# Autodesk Inventor assembly: 5A.00.02.01-IB-VTP-Final-Master-Assy
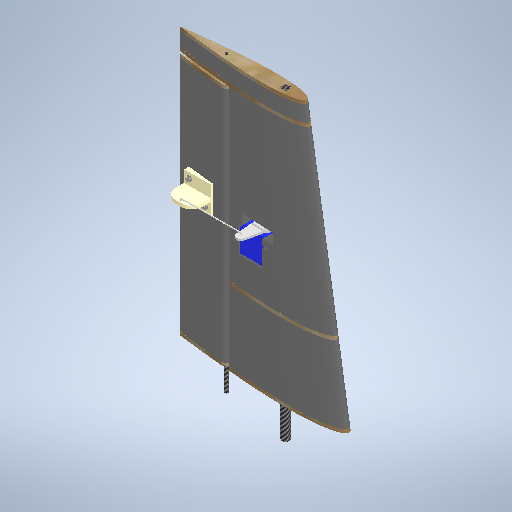
[picture p0: Inventor's stored thumbnail of the model, 512x512]
Saved by Autodesk Inventor 2025.2 (Build 292293000, 293)
## iProperties
Created: 2025-01-14
Part Number: 5A.00.02.01-IB-VTP-Final-Master-Assy
Document SubType Name: Assembly
Designer: inigo
Author: inigo
## Documents named in this file (27)
- C:\Users\inigo\OneDrive - University of Bristol\General - grp-Company A - AVDASI2 2024-25\Full Assembly\VTP\5A.00.02.01-IB-VTP-Final-Master-Assy.iam
- C:\Users\inigo\OneDrive - University of Bristol\General - grp-Company A - AVDASI2 2024-25\Full Assembly\VTP\5P.00.06.01-IB-VTP-Main-Spar.ipt
- C:\Users\inigo\OneDrive - University of Bristol\General - grp-Company A - AVDASI2 2024-25\Full Assembly\VTP\5P.00.08.01-IB-Rear-Spar.ipt
- C:\Users\inigo\OneDrive - University of Bristol\General - grp-Company A - AVDASI2 2024-25\Full Assembly\VTP\EMAX-09-MD Servo.ipt
- C:\Users\inigo\OneDrive - University of Bristol\General - grp-Company A - AVDASI2 2024-25\Full Assembly\VTP\5P.00.02.01-IB-VTP-Body-Final-Right-Second-Rib.ipt
- C:\Users\inigo\OneDrive - University of Bristol\General - grp-Company A - AVDASI2 2024-25\Full Assembly\VTP\5P.00.24.01-IB-VTP-Body-Final-Right-Top.ipt
- C:\Users\inigo\OneDrive - University of Bristol\General - grp-Company A - AVDASI2 2024-25\Full Assembly\VTP\5P.00.10.01-IB-VTP-Body-Final-Right-Main.ipt
- C:\Users\inigo\OneDrive - University of Bristol\General - grp-Company A - AVDASI2 2024-25\Full Assembly\VTP\5P.00.09.01-IB-VTP-Body-Final-Right-Bottom.ipt
- C:\Users\inigo\OneDrive - University of Bristol\General - grp-Company A - AVDASI2 2024-25\Full Assembly\VTP\5P.00.11.01-IB-VTP-Body-Final-Top-Rib.ipt
- C:\Users\inigo\OneDrive - University of Bristol\General - grp-Company A - AVDASI2 2024-25\Full Assembly\VTP\5P.00.12.01-IB-VTP-Body-Final-Middle-Rib.ipt
- C:\Users\inigo\OneDrive - University of Bristol\General - grp-Company A - AVDASI2 2024-25\Full Assembly\VTP\5P.00.13.01-IB-VTP-Body-Final-Bottom-Rib.ipt
- C:\Users\inigo\OneDrive - University of Bristol\General - grp-Company A - AVDASI2 2024-25\Full Assembly\VTP\5P.00.14.01-IB-VTP-Body-Final-Left-Top.ipt
- C:\Users\inigo\OneDrive - University of Bristol\General - grp-Company A - AVDASI2 2024-25\Full Assembly\VTP\5P.00.15.01-IB-VTP-Body-Final-Left-Bottom.ipt
- C:\Users\inigo\OneDrive - University of Bristol\General - grp-Company A - AVDASI2 2024-25\Full Assembly\VTP\5P.00.16.01-IB-VTP-Body-Final-Left-Main.ipt
- C:\Users\inigo\OneDrive - University of Bristol\General - grp-Company A - AVDASI2 2024-25\Full Assembly\VTP\5P.00.04.01-IB-VTP-Rudder-Right.ipt
- C:\Users\inigo\OneDrive - University of Bristol\General - grp-Company A - AVDASI2 2024-25\Full Assembly\VTP\5P.00.07.01-IB-VTP-Rudder-Bottom-Rib.ipt
- C:\Users\inigo\OneDrive - University of Bristol\General - grp-Company A - AVDASI2 2024-25\Full Assembly\VTP\5P.00.05.01-IB-VTP-Rudder-Left.ipt
- C:\Users\inigo\OneDrive - University of Bristol\General - grp-Company A - AVDASI2 2024-25\Full Assembly\VTP\5P.00.18.01-IB-VTP-Rudder-Top-Rib.ipt
- C:\Users\inigo\OneDrive - University of Bristol\General - grp-Company A - AVDASI2 2024-25\Full Assembly\VTP\5P.00.17.01-IB-VTP-Control-Horn.ipt
- C:\Users\inigo\OneDrive - University of Bristol\General - grp-Company A - AVDASI2 2024-25\Full Assembly\VTP\5P.00.19.01-IB-VTP-Servo-Horn.ipt
- C:\Users\inigo\OneDrive - University of Bristol\General - grp-Company A - AVDASI2 2024-25\Full Assembly\VTP\5P.00.20.01-IB-VTP-Control-Rod.ipt
- C:\Users\inigo\OneDrive - University of Bristol\General - grp-Company A - AVDASI2 2024-25\Full Assembly\VTP\5P.00.21.01-IB-VTP-Rudder-Backplate.ipt
- C:\Users\inigo\OneDrive - University of Bristol\General - grp-Company A - AVDASI2 2024-25\Full Assembly\VTP\5P.00.23.01-IB-VTP-Servo-Rear-Retaining-Rod.ipt
- C:\Users\inigo\OneDrive - University of Bristol\General - grp-Company A - AVDASI2 2024-25\Full Assembly\VTP\5P.00.22.01-IB-VTP-Servo-Front-Retaining-Rod.ipt
- C:\Users\inigo\Documents\Inventor\Content Center Files\R2024\en-US\ISO 4762(2)\ISO 4762 - M2 x 16ISO.ipt
- C:\Users\inigo\Documents\Inventor\Content Center Files\R2024\en-US\ISO 7089\ISO 7089 - 2 - 140 HV(1).ipt
- C:\Users\inigo\Documents\Inventor\Content Center Files\R2024\en-US\ISO 4032(2)\ISO 4032 - M2 - ISO.ipt
## Components (31 placed, 26 different names)
1. 5P.00.06.01-IB-VTP-Main-Spar:1 — Mate:1, Flush:1, Mate:3, Mate:6, Mate:9, Mate:12, Mate:14, Mate:16, Mate:18, Mate:20, Mate:29, Mate:51
2. 5P.00.08.01-IB-Rear-Spar:1 — Mate:2, Flush:2, Mate:4, Mate:7, Mate:10, Mate:31, Mate:33, Mate:35, Mate:37
3. EMAX-09-MD Servo:1 — Mate:22, Mate:23, Mate:24, Mate:25, Mate:27, Mate:48, Mate:49
4. 5P.00.02.01-IB-VTP-Body-Final-Second-Rib:1 — Mate:9, Mate:10, Mate:32, Mate:54, Mate:55, Mate:56
5. 5P.00.24.01-IB-VTP-Body-Final-Right-Top:1 — Mate:6, Mate:7, Mate:57, Mate:75
6. 5P.00.09.01-IB-VTP-Body-Final-Right-Bottom:1 — Mate:20, Mate:21, Mate:52
7. 5P.00.11.01-IB-VTP-Body-Final-Top-Rib:1 — Mate:1, Mate:2, Flush:1, Flush:2, Mate:74, Mate:75
8. 5P.00.12.01-IB-VTP-Body-Final-Middle-Rib:1 — Mate:14, Flush:3, Mate:15, Mate:17, Mate:21
9. 5P.00.13.01-IB-VTP-Body-Final-Bottom-Rib:1 — Mate:18, Mate:19, Flush:5
10. 5P.00.14.01-IB-VTP-Body-Final-Left-Top:1 — Mate:3, Mate:4, Mate:54, Angle:1, Mate:74
11. 5P.00.15.01-IB-VTP-Body-Final-Left-Bottom:1 — Mate:16, Flush:4, Mate:17, Mate:19, Flush:5, Mate:52
12. 5P.00.10.01-IB-VTP-Body-Final-Right-Main:1 — Mate:29, Flush:6, Mate:55
13. 5P.00.16.01-IB-VTP-Body-Final-Left-Main:1 — Mate:12, Flush:3, Mate:15, Flush:4, Mate:22, Mate:23, Mate:24, Mate:26, Mate:28, Flush:6, Mate:56, Angle:1
14. 5P.00.04.01-IB-VTP-Rudder-Right:1 — Mate:35, Mate:36, Mate:38, Mate:41, Mate:42, Mate:43, Mate:53
15. 5P.00.07.01-IB-VTP-Rudder-Bottom-Rib:1 — Mate:37, Mate:38, Mate:39
16. 5P.00.05.01-IB-VTP-Rudder-Left:1 — Mate:33, Mate:34, Mate:39, Mate:40, Mate:44, Mate:45, Mate:46, Mate:53
17. 5P.00.18.01-IB-VTP-Rudder-Top-Rib:1 — Mate:31, Mate:32, Mate:34, Mate:36, Mate:40
18. 5P.00.17.01-IB-VTP-Control-Horn:1 — Mate:41, Mate:42, Mate:43, Mate:47, Flush:7, Mate:62, Mate:63, Mate:64, Mate:65
19. 5P.00.20.01-IB-VTP-Control-Rod:1 — Mate:47, Mate:50, Flush:7
20. 5P.00.21.01-IB-VTP-Rudder-Backplate:1 — Mate:44, Mate:45, Mate:46, Mate:67, Mate:69
21. 5P.00.23.01-IB-VTP-Servo-Rear-Retaining-Rod:1 — Mate:25, Mate:26
22. 5P.00.22.01-IB-VTP-Servo-Front-Retaining-Rod:1 — Mate:27, Mate:28
23. 5P.00.19.01-IB-VTP-Servo-Horn:1 — Mate:48, Mate:49, Mate:50
24. ISO 4762 M2 x 16:1 — Mate:58, Mate:59, Mate:64, Mate:66, Mate:70
25. ISO 7089 2:1 — Mate:58, Mate:59, Mate:65
26. ISO 4762 M2 x 16:2 — Mate:62, Mate:68, Mate:72
27. ISO 7089 2:2 — Mate:63
28. ISO 7089 2:3 — Mate:66, Mate:67, Mate:71
29. ISO 7089 2:4 — Mate:68, Mate:69, Mate:73
30. ISO 4032 M2:1 — Mate:70, Mate:71
31. ISO 4032 M2:2 — Mate:72, Mate:73
## Relationships (78: Mate 70, Flush 7, Angle 1)
- Mate:1: 5P.00.06.01-IB-VTP-Main-Spar:1 ↔ 5P.00.11.01-IB-VTP-Body-Final-Top-Rib:1
- Mate:2: 5P.00.08.01-IB-Rear-Spar:1 ↔ 5P.00.11.01-IB-VTP-Body-Final-Top-Rib:1
- Flush:1: 5P.00.06.01-IB-VTP-Main-Spar:1 ↔ 5P.00.11.01-IB-VTP-Body-Final-Top-Rib:1
- Flush:2: 5P.00.08.01-IB-Rear-Spar:1 ↔ 5P.00.11.01-IB-VTP-Body-Final-Top-Rib:1
- Mate:3: 5P.00.06.01-IB-VTP-Main-Spar:1 ↔ 5P.00.14.01-IB-VTP-Body-Final-Left-Top:1
- Mate:4: 5P.00.08.01-IB-Rear-Spar:1 ↔ 5P.00.14.01-IB-VTP-Body-Final-Left-Top:1
- Mate:6: 5P.00.06.01-IB-VTP-Main-Spar:1 ↔ 5P.00.24.01-IB-VTP-Body-Final-Right-Top:1
- Mate:7: 5P.00.08.01-IB-Rear-Spar:1 ↔ 5P.00.24.01-IB-VTP-Body-Final-Right-Top:1
- Mate:9: 5P.00.06.01-IB-VTP-Main-Spar:1 ↔ 5P.00.02.01-IB-VTP-Body-Final-Second-Rib:1
- Mate:10: 5P.00.08.01-IB-Rear-Spar:1 ↔ 5P.00.02.01-IB-VTP-Body-Final-Second-Rib:1
- Mate:12: 5P.00.06.01-IB-VTP-Main-Spar:1 ↔ 5P.00.16.01-IB-VTP-Body-Final-Left-Main:1
- Mate:14: 5P.00.06.01-IB-VTP-Main-Spar:1 ↔ 5P.00.12.01-IB-VTP-Body-Final-Middle-Rib:1
- Flush:3: 5P.00.12.01-IB-VTP-Body-Final-Middle-Rib:1 ↔ 5P.00.16.01-IB-VTP-Body-Final-Left-Main:1
- Mate:15: 5P.00.12.01-IB-VTP-Body-Final-Middle-Rib:1 ↔ 5P.00.16.01-IB-VTP-Body-Final-Left-Main:1
- Mate:16: 5P.00.06.01-IB-VTP-Main-Spar:1 ↔ 5P.00.15.01-IB-VTP-Body-Final-Left-Bottom:1
- Flush:4: 5P.00.15.01-IB-VTP-Body-Final-Left-Bottom:1 ↔ 5P.00.16.01-IB-VTP-Body-Final-Left-Main:1
- Mate:17: 5P.00.12.01-IB-VTP-Body-Final-Middle-Rib:1 ↔ 5P.00.15.01-IB-VTP-Body-Final-Left-Bottom:1
- Mate:18: 5P.00.06.01-IB-VTP-Main-Spar:1 ↔ 5P.00.13.01-IB-VTP-Body-Final-Bottom-Rib:1
- Mate:19: 5P.00.13.01-IB-VTP-Body-Final-Bottom-Rib:1 ↔ 5P.00.15.01-IB-VTP-Body-Final-Left-Bottom:1
- Flush:5: 5P.00.13.01-IB-VTP-Body-Final-Bottom-Rib:1 ↔ 5P.00.15.01-IB-VTP-Body-Final-Left-Bottom:1
- Mate:20: 5P.00.06.01-IB-VTP-Main-Spar:1 ↔ 5P.00.09.01-IB-VTP-Body-Final-Right-Bottom:1
- Mate:21: 5P.00.09.01-IB-VTP-Body-Final-Right-Bottom:1 ↔ 5P.00.12.01-IB-VTP-Body-Final-Middle-Rib:1
- Mate:22: EMAX-09-MD Servo:1 ↔ 5P.00.16.01-IB-VTP-Body-Final-Left-Main:1
- Mate:23: EMAX-09-MD Servo:1 ↔ 5P.00.16.01-IB-VTP-Body-Final-Left-Main:1
- Mate:24: EMAX-09-MD Servo:1 ↔ 5P.00.16.01-IB-VTP-Body-Final-Left-Main:1
- Mate:25: EMAX-09-MD Servo:1 ↔ 5P.00.23.01-IB-VTP-Servo-Rear-Retaining-Rod:1
- Mate:26: 5P.00.16.01-IB-VTP-Body-Final-Left-Main:1 ↔ 5P.00.23.01-IB-VTP-Servo-Rear-Retaining-Rod:1
- Mate:27: EMAX-09-MD Servo:1 ↔ 5P.00.22.01-IB-VTP-Servo-Front-Retaining-Rod:1
- Mate:28: 5P.00.16.01-IB-VTP-Body-Final-Left-Main:1 ↔ 5P.00.22.01-IB-VTP-Servo-Front-Retaining-Rod:1
- Mate:29: 5P.00.06.01-IB-VTP-Main-Spar:1 ↔ 5P.00.10.01-IB-VTP-Body-Final-Right-Main:1
- Flush:6: 5P.00.10.01-IB-VTP-Body-Final-Right-Main:1 ↔ 5P.00.16.01-IB-VTP-Body-Final-Left-Main:1
- Mate:31: 5P.00.08.01-IB-Rear-Spar:1 ↔ 5P.00.18.01-IB-VTP-Rudder-Top-Rib:1
- Mate:32 (2 mm): 5P.00.02.01-IB-VTP-Body-Final-Second-Rib:1 ↔ 5P.00.18.01-IB-VTP-Rudder-Top-Rib:1
- Mate:33: 5P.00.08.01-IB-Rear-Spar:1 ↔ 5P.00.05.01-IB-VTP-Rudder-Left:1
- Mate:34: 5P.00.05.01-IB-VTP-Rudder-Left:1 ↔ 5P.00.18.01-IB-VTP-Rudder-Top-Rib:1
- Mate:35: 5P.00.08.01-IB-Rear-Spar:1 ↔ 5P.00.04.01-IB-VTP-Rudder-Right:1
- Mate:36: 5P.00.04.01-IB-VTP-Rudder-Right:1 ↔ 5P.00.18.01-IB-VTP-Rudder-Top-Rib:1
- Mate:37: 5P.00.08.01-IB-Rear-Spar:1 ↔ 5P.00.07.01-IB-VTP-Rudder-Bottom-Rib:1
- Mate:38: 5P.00.04.01-IB-VTP-Rudder-Right:1 ↔ 5P.00.07.01-IB-VTP-Rudder-Bottom-Rib:1
- Mate:39: 5P.00.07.01-IB-VTP-Rudder-Bottom-Rib:1 ↔ 5P.00.05.01-IB-VTP-Rudder-Left:1
- Mate:40: 5P.00.05.01-IB-VTP-Rudder-Left:1 ↔ 5P.00.18.01-IB-VTP-Rudder-Top-Rib:1
- Mate:41: 5P.00.04.01-IB-VTP-Rudder-Right:1 ↔ 5P.00.17.01-IB-VTP-Control-Horn:1
- Mate:42: 5P.00.04.01-IB-VTP-Rudder-Right:1 ↔ 5P.00.17.01-IB-VTP-Control-Horn:1
- Mate:43 (-6 mm): 5P.00.04.01-IB-VTP-Rudder-Right:1 ↔ 5P.00.17.01-IB-VTP-Control-Horn:1
- Mate:44: 5P.00.05.01-IB-VTP-Rudder-Left:1 ↔ 5P.00.21.01-IB-VTP-Rudder-Backplate:1
- Mate:45 (-6 mm): 5P.00.05.01-IB-VTP-Rudder-Left:1 ↔ 5P.00.21.01-IB-VTP-Rudder-Backplate:1
- Mate:46: 5P.00.05.01-IB-VTP-Rudder-Left:1 ↔ 5P.00.21.01-IB-VTP-Rudder-Backplate:1
- Mate:47: 5P.00.17.01-IB-VTP-Control-Horn:1 ↔ 5P.00.20.01-IB-VTP-Control-Rod:1
- Mate:48: EMAX-09-MD Servo:1 ↔ 5P.00.19.01-IB-VTP-Servo-Horn:1
- Mate:49: EMAX-09-MD Servo:1 ↔ 5P.00.19.01-IB-VTP-Servo-Horn:1
- Mate:50: 5P.00.20.01-IB-VTP-Control-Rod:1 ↔ 5P.00.19.01-IB-VTP-Servo-Horn:1
- Flush:7 (-1 mm): 5P.00.17.01-IB-VTP-Control-Horn:1 ↔ 5P.00.20.01-IB-VTP-Control-Rod:1
- Mate:51: 5P.00.06.01-IB-VTP-Main-Spar:1
- Mate:52: 5P.00.09.01-IB-VTP-Body-Final-Right-Bottom:1 ↔ 5P.00.15.01-IB-VTP-Body-Final-Left-Bottom:1
- Mate:53: 5P.00.04.01-IB-VTP-Rudder-Right:1 ↔ 5P.00.05.01-IB-VTP-Rudder-Left:1
- Mate:54: 5P.00.02.01-IB-VTP-Body-Final-Second-Rib:1 ↔ 5P.00.14.01-IB-VTP-Body-Final-Left-Top:1
- Mate:55: 5P.00.02.01-IB-VTP-Body-Final-Second-Rib:1 ↔ 5P.00.10.01-IB-VTP-Body-Final-Right-Main:1
- Mate:56: 5P.00.02.01-IB-VTP-Body-Final-Second-Rib:1 ↔ 5P.00.16.01-IB-VTP-Body-Final-Left-Main:1
- Angle:1 (90 deg): 5P.00.14.01-IB-VTP-Body-Final-Left-Top:1 ↔ 5P.00.16.01-IB-VTP-Body-Final-Left-Main:1
- Mate:57: 5P.00.24.01-IB-VTP-Body-Final-Right-Top:1
- Mate:58: ISO 4762 M2 x 16:1 ↔ ISO 7089 2:1
- Mate:59: ISO 4762 M2 x 16:1 ↔ ISO 7089 2:1
- [Mate]: ISO 4762 M2 x 16:2 ↔ ISO 7089 2:2
- [Mate]: ISO 4762 M2 x 16:2 ↔ ISO 7089 2:2
- Mate:62: 5P.00.17.01-IB-VTP-Control-Horn:1 ↔ ISO 4762 M2 x 16:2
- Mate:63: 5P.00.17.01-IB-VTP-Control-Horn:1 ↔ ISO 7089 2:2
- Mate:64: 5P.00.17.01-IB-VTP-Control-Horn:1 ↔ ISO 4762 M2 x 16:1
- Mate:65: 5P.00.17.01-IB-VTP-Control-Horn:1 ↔ ISO 7089 2:1
- Mate:66: ISO 4762 M2 x 16:1 ↔ ISO 7089 2:3
- Mate:67: 5P.00.21.01-IB-VTP-Rudder-Backplate:1 ↔ ISO 7089 2:3
- Mate:68: ISO 4762 M2 x 16:2 ↔ ISO 7089 2:4
- Mate:69: 5P.00.21.01-IB-VTP-Rudder-Backplate:1 ↔ ISO 7089 2:4
- Mate:70: ISO 4762 M2 x 16:1 ↔ ISO 4032 M2:1
- Mate:71: ISO 7089 2:3 ↔ ISO 4032 M2:1
- Mate:72: ISO 4762 M2 x 16:2 ↔ ISO 4032 M2:2
- Mate:73: ISO 7089 2:4 ↔ ISO 4032 M2:2
- Mate:74: 5P.00.11.01-IB-VTP-Body-Final-Top-Rib:1 ↔ 5P.00.14.01-IB-VTP-Body-Final-Left-Top:1
- Mate:75: 5P.00.24.01-IB-VTP-Body-Final-Right-Top:1 ↔ 5P.00.11.01-IB-VTP-Body-Final-Top-Rib:1
## Named parameters: d176_d174 = 0 mm, d177_d175 = 0 mm
